# Autodesk Inventor assembly: Leg Right v0.1
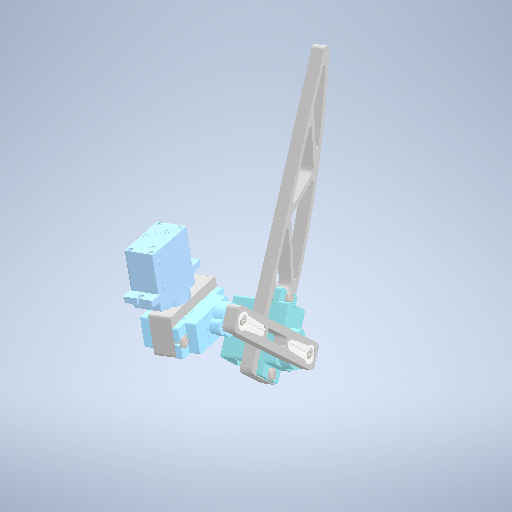
[picture p0: Inventor's stored thumbnail of the model, 512x512]
Saved by Autodesk Inventor 2025 (Build 290162000, 162)
## iProperties
Created: 2024-06-04
Part Number: Leg Right v0.1
Document SubType Name: Assembly
Designer: sgols
Author: sgols
## iProperties of the stored document SG90 - Micro Servo 9g - Tower Pro.1.ipt
Created: 2017-11-11
Part Number: SG90 - Micro Servo 9g - Tower Pro.1
Material: solidworks materials|PVC Rígido
Document SubType Name: Modeling
Designer: sgols
Density: 1.3 g/cm^3
Appearance: white medium gloss plastic
Sending System: SolidWorks 2016
Last Author: mathe
Last Saved: 2017-11-11
Quantidade: 01
Peso: 9.16
Material: PVC Rígido
Projetista: Matheus A. Frasson
Data do Projeto: 00/00/0000
Revisão: Matheus A. Frasson
Aprovação: Matheus A. Frasson
Data de Aprovação: 00/00/0000
Custo Total: 0.00
Author: Matheus A. Frasson
Comments: Propriedade de: Matheus A. Frasson E-mail: matheusprojetos1@gmail.com
## Documents named in this file (9)
- C:\git\hexapod\mechanics\Leg Right v0.1.iam
- C:\git\hexapod\mechanics\Femur v0.1.ipt
- C:\git\hexapod\mechanics\Foot v0.1.ipt
- C:\git\hexapod\mechanics\Hip v0.1.ipt
- **C:\git\hexapod\mechanics\Leg Right v0.1.iam*LocalDocs*xAaaaa2baAaaaaaaaAaaaqdmzIg*SG90 - Micro Servo 9g - Tower Pro.1.ipt
- C:\git\hexapod\mechanics\Servos\Micro Servo 9g\SG90 - Micro Servo 9g - Tower Pro.2\SG90 - Micro Servo 9g - Tower Pro.2.ipt
- C:\git\hexapod\mechanics\Servos\Micro Servo 9g\SG90 - Micro Servo 9g - Tower Pro.5\SG90 - Micro Servo 9g - Tower Pro.5.ipt
- C:\git\hexapod\mechanics\Servos\Micro Servo 9g\SG90 - Micro Servo 9g - Tower Pro.6\SG90 - Micro Servo 9g - Tower Pro.6.ipt
- C:\git\hexapod\mechanics\Servos\Micro Servo 9g\SG90 - Micro Servo 9g - Tower Pro.1.SLDPRT
## Components (16 placed, 9 different names)
1. Femur v0.1:1 — Insert:2, Mate:2, Insert:3, Mate:3
2. Foot v0.1:1 — Mate:7, Mate:8, Mate:9
3. Hip v0.1:1 — Mate:1, Mate:4, Mate:5, Mate:6, Mate:10, Mate:11
4. SG90 - Micro Servo 9g - Tower Pro.5:1 — Insert:10
5. SG90 - Micro Servo 9g - Tower Pro.5:2 — Insert:8
6. SG90 - Micro Servo 9g - Tower Pro.5:3 — Insert:7
7. SG90 - Micro Servo 9g - Tower Pro.5:4 — Insert:9
8. SG90 - Micro Servo 9g - Tower Pro.6:1 — Insert:6
9. SG90 - Micro Servo 9g - Tower Pro.6:2 — Insert:4
10. SG90 - Micro Servo 9g - Tower Pro.6:3 — Insert:5
11. Servo Hip — Rotational:1
12. Servo Femur — Mate:4, Mate:5, Mate:6, Rotational:2, Insert:9, Insert:10
13. Servo Foot — Mate:7, Mate:8, Mate:9, Rotational:3, Insert:7, Insert:8
14. SG90 - Micro Servo 9g - Tower Pro.2:3 — Mate:1, Rotational:1, Insert:6, Mate:10, Mate:11
15. SG90 - Micro Servo 9g - Tower Pro.2:2 — Insert:2, Mate:2, Rotational:2, Insert:5
16. SG90 - Micro Servo 9g - Tower Pro.2:1 — Insert:3, Mate:3, Rotational:3, Insert:4
## Relationships (23: Mate 11, Insert 9, RevoluteJoint 3)
- Mate:1: Hip v0.1:1 ↔ SG90 - Micro Servo 9g - Tower Pro.2:3
- Insert:2: Femur v0.1:1 ↔ SG90 - Micro Servo 9g - Tower Pro.2:2
- Mate:2: Femur v0.1:1 ↔ SG90 - Micro Servo 9g - Tower Pro.2:2
- Insert:3: Femur v0.1:1 ↔ SG90 - Micro Servo 9g - Tower Pro.2:1
- Mate:3: Femur v0.1:1 ↔ SG90 - Micro Servo 9g - Tower Pro.2:1
- Rotational:1 [RevoluteJoint]: Servo Hip ↔ SG90 - Micro Servo 9g - Tower Pro.2:3
- Mate:4: Hip v0.1:1 ↔ Servo Femur
- Mate:5: Hip v0.1:1 ↔ Servo Femur
- Mate:6: Hip v0.1:1 ↔ Servo Femur
- Mate:7: Foot v0.1:1 ↔ Servo Foot
- Mate:8: Foot v0.1:1 ↔ Servo Foot
- Mate:9: Foot v0.1:1 ↔ Servo Foot
- Rotational:2 [RevoluteJoint]: Servo Femur ↔ SG90 - Micro Servo 9g - Tower Pro.2:2
- Rotational:3 [RevoluteJoint]: Servo Foot ↔ SG90 - Micro Servo 9g - Tower Pro.2:1
- Insert:4: SG90 - Micro Servo 9g - Tower Pro.6:2 ↔ SG90 - Micro Servo 9g - Tower Pro.2:1
- Insert:5: SG90 - Micro Servo 9g - Tower Pro.6:3 ↔ SG90 - Micro Servo 9g - Tower Pro.2:2
- Insert:6: SG90 - Micro Servo 9g - Tower Pro.6:1 ↔ SG90 - Micro Servo 9g - Tower Pro.2:3
- Mate:10: Hip v0.1:1 ↔ SG90 - Micro Servo 9g - Tower Pro.2:3
- Mate:11: Hip v0.1:1 ↔ SG90 - Micro Servo 9g - Tower Pro.2:3
- Insert:7: SG90 - Micro Servo 9g - Tower Pro.5:3 ↔ Servo Foot
- Insert:8: SG90 - Micro Servo 9g - Tower Pro.5:2 ↔ Servo Foot
- Insert:9: SG90 - Micro Servo 9g - Tower Pro.5:4 ↔ Servo Femur
- Insert:10: SG90 - Micro Servo 9g - Tower Pro.5:1 ↔ Servo Femur
